# Autodesk Inventor assembly: am-1238+Collar+Clamp,+0.5''+Hex+Bore,+Aluminum
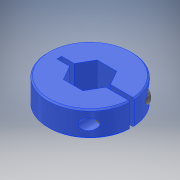
[picture p0: Inventor's stored thumbnail of the model, 180x180]
Saved by Autodesk Inventor 2018 (Build 220112000, 112)
## iProperties
Created: 2017-06-08
Part Number: am-1238+Collar+Clamp,+0.5''+Hex+Bore,+Aluminum
Document SubType Name: Assembly
Designer: maste
Author: maste
Revision Number: ANY
## Documents named in this file (3)
- F:\Summer Drive Base V1\Summer Drivebase\am-1238+Collar+Clamp,+0.5''+Hex+Bore,+Aluminum.iam
- F:\Summer Drive Base V1\Summer Drivebase\am-1238 Clamp Only.ipt
- F:\Summer Drive Base V1\Summer Drivebase\am-1238 Screw Only_91251A194.ipt
## Components (2 placed, 2 different names)
1. am-1238 Clamp Only_1 — Mate:1, Mate:2, Rotation:1
2. am-1238 Screw Only_91251A194_2 — Mate:1, Mate:2, Rotation:1
## Relationships (3: Mate 2, RelateRotation 1)
- Mate:1: am-1238 Clamp Only_1 ↔ am-1238 Screw Only_91251A194_2
- Mate:2: am-1238 Clamp Only_1 ↔ am-1238 Screw Only_91251A194_2
- Rotation:1 [RelateRotation] (1 ul): am-1238 Clamp Only_1 ↔ am-1238 Screw Only_91251A194_2
